# Autodesk Inventor assembly: механизм открывания форточкой
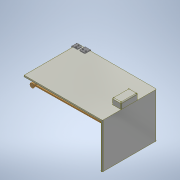
[picture p0: Inventor's stored thumbnail of the model, 180x180]
Saved by Autodesk Inventor 2021 (Build 250183000, 183)
## iProperties
Created: 2023-02-16
Part Number: механизм открывания форточкой
Document SubType Name: Assembly
Designer: Tasya
Author: Tasya
## Documents named in this file (10)
- C:\Users\Tasya\Desktop\теплица\3D модели\Сборки iam\механизм открывания форточкой.iam
- C:\Users\Tasya\Desktop\теплица\форточка\основание форточки.ipt
- C:\Users\Tasya\Desktop\теплица\форточка\коробка + сервак.iam
- C:\Users\Tasya\Desktop\теплица\grabcad\Switch on off.ipt
- C:\Users\Tasya\Desktop\теплица\grabcad\Wemos_D1_mini.ipt
- C:\Users\Tasya\Desktop\теплица\grabcad\Датчик тока acs712.iam
- C:\Users\Tasya\Desktop\теплица\grabcad\конденсатор.ipt
- C:\Users\Tasya\Desktop\теплица\форточка\кронштейн.ipt
- C:\Users\Tasya\Desktop\теплица\форточка\вал.ipt
- C:\Users\Tasya\Desktop\теплица\форточка\втулка.ipt
## Components (9 placed, 9 different names)
1. основание форточки:1 — Заподлицо:1, Совмещение:1, Заподлицо:2, Совмещение:3, Совмещение:10
2. коробка + сервак:1 [sub-assembly] — Заподлицо:1, Совмещение:1, Заподлицо:2, Совмещение:2, Совмещение:4, Совмещение:8, Совмещение:9
3. Switch on off:1 — Совмещение:10
4. Wemos_D1_mini:1
5. Датчик тока acs712:1 [sub-assembly]
6. конденсатор:1
7. кронштейн:1 — Совмещение:2, Совмещение:3, Совмещение:4
8. вал:1 — Совмещение:5, Совмещение:6, Совмещение:7
9. втулка:1 — Совмещение:5, Совмещение:6, Совмещение:7, Совмещение:8, Совмещение:9
## Relationships (12: Mate 10, Flush 2)
- Заподлицо:1 [Flush]: основание форточки:1 ↔ коробка + сервак:1
- Совмещение:1 [Mate]: основание форточки:1 ↔ коробка + сервак:1
- Заподлицо:2 [Flush]: основание форточки:1 ↔ коробка + сервак:1
- Совмещение:2 [Mate]: коробка + сервак:1 ↔ кронштейн:1
- Совмещение:3 [Mate]: основание форточки:1 ↔ кронштейн:1
- Совмещение:4 [Mate]: коробка + сервак:1 ↔ кронштейн:1
- Совмещение:5 [Mate]: вал:1 ↔ втулка:1
- Совмещение:6 [Mate]: вал:1 ↔ втулка:1
- Совмещение:7 [Mate]: вал:1 ↔ втулка:1
- Совмещение:8 [Mate]: коробка + сервак:1 ↔ втулка:1
- Совмещение:9 [Mate]: коробка + сервак:1 ↔ втулка:1
- Совмещение:10 [Mate]: основание форточки:1 ↔ Switch on off:1
